# Autodesk Inventor assembly: winchAssembly
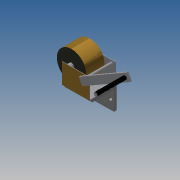
[picture p0: Inventor's stored thumbnail of the model, 180x180]
Saved by Autodesk Inventor 2014 SP1 (Build 180222100, 222)
## iProperties
Company: HERA Project
Created: 2013-12-16
Part Number: winchAssembly
Document SubType Name: Assembly
Designer: Dave
Author: David DeBoer
Title: Winch
## Documents named in this file (3)
- C:\Users\Dave\Desktop\hera-cad\support\winchAssembly.iam
- C:\Users\Dave\Desktop\hera-cad\smallParts\winch.ipt
- C:\Users\Dave\Desktop\hera-cad\smallParts\thickRightAngle.ipt
## Components (2 placed, 2 different names)
1. winch:1 — Insert:1
2. thickRightAngle:1 — Insert:1
## Relationships (1: Insert 1)
- Insert:1: winch:1 ↔ thickRightAngle:1
